# Autodesk Inventor assembly: ASY GBK правая стенка
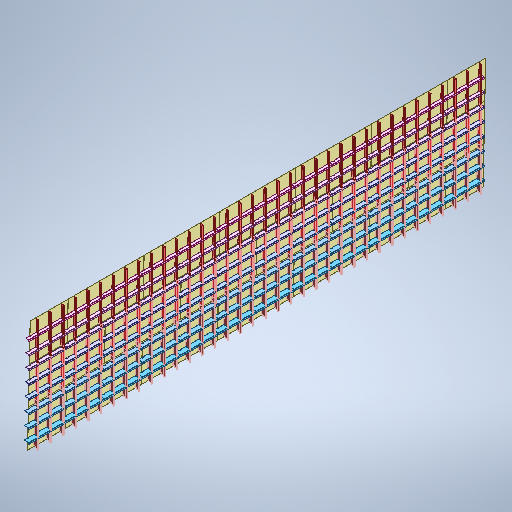
[picture p0: Inventor's stored thumbnail of the model, 512x512]
Saved by Autodesk Inventor 2026.2 (Build 302298000, 298)
## iProperties
Created: 2026-05-20
Part Number: ASY GBK правая стенка
Document SubType Name: Assembly
Designer: admin
Mass: 4.44159e+06 g
Surface Area: 2.86879e+06 cm^2
Volume: 565808 cm^3
Density: 7.85 g/cm^3
Author: admin
## Documents named in this file (6)
- C:\Users\admin\Documents\Inventor\GBK-Gubkinskiy\ASY GBK правая стенка.iam
- C:\Users\admin\Documents\Inventor\GBK-Gubkinskiy\01 ASY GBK wall shield 1.1.1.iam
- C:\Users\admin\Documents\Inventor\GBK-Gubkinskiy\02 ASY GBK wall shield 1.1.2.iam
- C:\Users\admin\Documents\Inventor\GBK-Gubkinskiy\04 ASY GBK wall shield 1.2.4.iam
- C:\Users\admin\Documents\Inventor\GBK-Gubkinskiy\07 ASY GBK wall shield 1.3.1.iam
- C:\Users\admin\Documents\Inventor\GBK-Gubkinskiy\08 ASY GBK wall shield 1.3.8.iam
## Components (20 placed, 6 different names)
1. 01 ASY GBK wall shield 1.1.1.iam:1 [sub-assembly] — Flush:1, Mate:1, Mate:2
2. 02 ASY GBK wall shield 1.1.2:1 [sub-assembly]
3. 04 ASY GBK wall shield 1.2.4:1 [sub-assembly]
4. 07 ASY GBK wall shield 1.3.1:1 [sub-assembly]
5. 08 ASY GBK wall shield 1.3.8:1 [sub-assembly]
6. 08 ASY GBK wall shield 1.3.8:2 [sub-assembly]
7. 08 ASY GBK wall shield 1.3.8:3 [sub-assembly]
8. 08 ASY GBK wall shield 1.3.8:4 [sub-assembly]
9. 08 ASY GBK wall shield 1.3.8:5 [sub-assembly]
10. 04 ASY GBK wall shield 1.2.4:2 [sub-assembly]
11. 04 ASY GBK wall shield 1.2.4:3 [sub-assembly]
12. 04 ASY GBK wall shield 1.2.4:4 [sub-assembly]
13. 04 ASY GBK wall shield 1.2.4:5 [sub-assembly]
14. 04 ASY GBK wall shield 1.2.4:6 [sub-assembly]
15. 02 ASY GBK wall shield 1.1.2:2 [sub-assembly]
16. 02 ASY GBK wall shield 1.1.2:3 [sub-assembly]
17. 02 ASY GBK wall shield 1.1.2:4 [sub-assembly]
18. 02 ASY GBK wall shield 1.1.2:5 [sub-assembly]
19. 01 ASY GBK wall shield 1.1.1:2 [sub-assembly]
20. 07 ASY GBK wall shield 1.3.1:2 [sub-assembly]
## Relationships (22: WeldJoint 19, Mate 2, Flush 1)
- [WeldJoint] (1 mm): 01 ASY GBK wall shield 1.1.1.iam:1 ↔ 02 ASY GBK wall shield 1.1.2:1
- [WeldJoint]: 01 ASY GBK wall shield 1.1.1.iam:1 ↔ 04 ASY GBK wall shield 1.2.4:1
- [WeldJoint]: 04 ASY GBK wall shield 1.2.4:1 ↔ 07 ASY GBK wall shield 1.3.1:1
- [WeldJoint] (1 mm): 07 ASY GBK wall shield 1.3.1:1 ↔ 08 ASY GBK wall shield 1.3.8:1
- [WeldJoint] (1 mm): 08 ASY GBK wall shield 1.3.8:1 ↔ 08 ASY GBK wall shield 1.3.8:2
- [WeldJoint] (1 mm): 08 ASY GBK wall shield 1.3.8:2 ↔ 08 ASY GBK wall shield 1.3.8:3
- [WeldJoint] (1 mm): 08 ASY GBK wall shield 1.3.8:3 ↔ 08 ASY GBK wall shield 1.3.8:4
- [WeldJoint] (1 mm): 08 ASY GBK wall shield 1.3.8:4 ↔ 08 ASY GBK wall shield 1.3.8:5
- [WeldJoint] (1 mm): 04 ASY GBK wall shield 1.2.4:1 ↔ 04 ASY GBK wall shield 1.2.4:2
- [WeldJoint] (1 mm): 04 ASY GBK wall shield 1.2.4:2 ↔ 04 ASY GBK wall shield 1.2.4:3
- [WeldJoint] (1 mm): 04 ASY GBK wall shield 1.2.4:3 ↔ 04 ASY GBK wall shield 1.2.4:4
- [WeldJoint] (1 mm): 04 ASY GBK wall shield 1.2.4:4 ↔ 04 ASY GBK wall shield 1.2.4:5
- [WeldJoint] (1 mm): 04 ASY GBK wall shield 1.2.4:5 ↔ 04 ASY GBK wall shield 1.2.4:6
- [WeldJoint] (1 mm): 02 ASY GBK wall shield 1.1.2:1 ↔ 02 ASY GBK wall shield 1.1.2:2
- [WeldJoint] (1 mm): 02 ASY GBK wall shield 1.1.2:2 ↔ 02 ASY GBK wall shield 1.1.2:3
- [WeldJoint] (1 mm): 02 ASY GBK wall shield 1.1.2:3 ↔ 02 ASY GBK wall shield 1.1.2:4
- [WeldJoint] (1 mm): 02 ASY GBK wall shield 1.1.2:4 ↔ 02 ASY GBK wall shield 1.1.2:5
- [WeldJoint] (1 mm): 02 ASY GBK wall shield 1.1.2:5 ↔ 01 ASY GBK wall shield 1.1.1:2
- [WeldJoint] (1 mm): 08 ASY GBK wall shield 1.3.8:5 ↔ 07 ASY GBK wall shield 1.3.1:2
- Flush:1: 01 ASY GBK wall shield 1.1.1.iam:1
- Mate:1: 01 ASY GBK wall shield 1.1.1.iam:1
- Mate:2: 01 ASY GBK wall shield 1.1.1.iam:1
## Named parameters: Зазор_по_горизонту = 1 mm
